# Autodesk Inventor assembly: LaptopTopDisplay
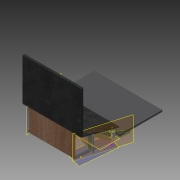
[picture p0: Inventor's stored thumbnail of the model, 180x180]
Saved by Autodesk Inventor 2017 (Build 210142000, 142)
## iProperties
Created: 2018-10-12
Part Number: LaptopTopDisplay
Document SubType Name: Assembly
Designer: ari
Author: ari
## Documents named in this file (8)
- C:\Users\ari\Documents\Inventor\LaptopTopDisplay\LaptopTopDisplay.iam
- C:\Users\ari\Documents\Inventor\LaptopTopDisplay\laptop.ipt
- C:\Users\ari\Documents\Inventor\LaptopTopDisplay\extDisplay.ipt
- C:\Users\ari\Documents\Inventor\LaptopTopDisplay\Stand.ipt
- C:\Users\ari\Documents\Inventor\LaptopTopDisplay\Stand_MIR.ipt
- C:\Users\ari\Documents\Inventor\LaptopTopDisplay\stand_bottom.ipt
- C:\Users\ari\Documents\Inventor\LaptopTopDisplay\brace_1.ipt
- C:\Users\ari\Documents\Inventor\LaptopTopDisplay\brace_2.ipt
## Components (7 placed, 7 different names)
1. laptop:1 — Mate:2, Mate:3, Angle:1, Mate:17, Mate:18, Flush:2
2. extDisplay:1 — Mate:2, Mate:3, Angle:1, Flush:1, Mate:4, Mate:7, Mate:8, Mate:14
3. Stand:1 — Mate:4, Mate:17, Mate:18, Mate:21
4. Stand_MIR:1 — Mate:7, Mate:8, Mate:14, Mate:19, Mate:20
5. stand_bottom:1 — Flush:2, Mate:19, Mate:20, Mate:21
6. brace_1:1
7. brace_2:1
## Relationships (14: Mate 11, Flush 2, Angle 1)
- Mate:2 (7 mm): laptop:1 ↔ extDisplay:1
- Mate:3 (-25 mm): laptop:1 ↔ extDisplay:1
- Angle:1 (165 deg): laptop:1 ↔ extDisplay:1
- Flush:1: extDisplay:1
- Mate:4 (0.5 mm): extDisplay:1 ↔ Stand:1
- Mate:7 (0.5 mm): extDisplay:1 ↔ Stand_MIR:1
- Mate:8 (0.5 mm): extDisplay:1 ↔ Stand_MIR:1
- Mate:14 (0.5 mm): extDisplay:1 ↔ Stand_MIR:1
- Mate:17: laptop:1 ↔ Stand:1
- Mate:18: laptop:1 ↔ Stand:1
- Flush:2: laptop:1 ↔ stand_bottom:1
- Mate:19: Stand_MIR:1 ↔ stand_bottom:1
- Mate:20: Stand_MIR:1 ↔ stand_bottom:1
- Mate:21: Stand:1 ↔ stand_bottom:1
